# Autodesk Inventor assembly: bike-rack-assembly
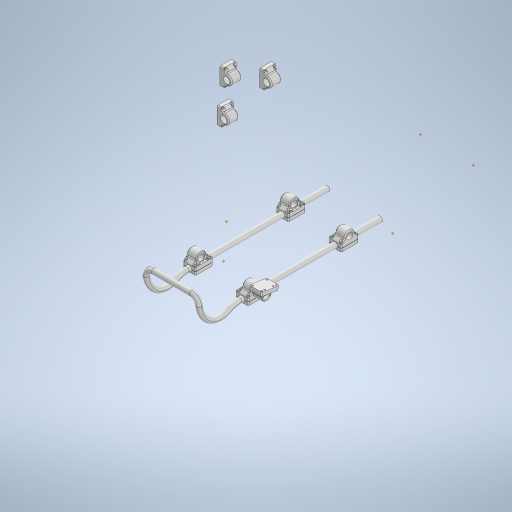
[picture p0: Inventor's stored thumbnail of the model, 512x512]
Saved by Autodesk Inventor 2024.1 (Build 281209000, 209)
## iProperties
Created: 2025-08-15
Part Number: bike-rack-assembly
Document SubType Name: Assembly
Designer: iwheard
Author: iwheard
## Documents named in this file (5)
- C:\Users\iwheard\Documents\0004-CAD\3D-cad-main\bike-rack\bike-rack-assembly.iam
- C:\Users\iwheard\Documents\0004-CAD\3D-cad-main\bike-rack\bike-rack.ipt
- C:\Users\iwheard\Documents\0004-CAD\3D-cad-main\h6-case\rack-mounts.ipt
- C:\Users\iwheard\Documents\0004-CAD\3D-cad-main\h6-case\rack-mounts_MIR.ipt
- C:\Users\iwheard\Documents\0004-CAD\3D-cad-main\h6-case\bucket-mounts.ipt
## Components (9 placed, 4 different names)
1. bike-rack:1 — Flush:1, Mate:1, Flush:2, Tangent:1, Tangent:2
2. rack-mounts:1 — Flush:1, Mate:1, Flush:2, Mate:2, Flush:3, Flush:4, Insert:1, Mate:4
3. rack-mounts:2 — Mate:2, Flush:3, Flush:4
4. rack-mounts_MIR:1 — Flush:5, Flush:6, Mate:3
5. rack-mounts_MIR:2 — Flush:5, Flush:6, Mate:3
6. bucket-mounts:1
7. bucket-mounts:2
8. bucket-mounts:3 — Insert:1, Mate:4
9. bucket-mounts:4
## Relationships (16: Flush 6, Mate 4, Angle 2, Tangent 2, Symmetry 1, Insert 1)
- Flush:1: bike-rack:1 ↔ rack-mounts:1
- Mate:1: bike-rack:1 ↔ rack-mounts:1
- Flush:2 (-240 mm): bike-rack:1 ↔ rack-mounts:1
- Mate:2 (150 mm): rack-mounts:1 ↔ rack-mounts:2
- Flush:3: rack-mounts:1 ↔ rack-mounts:2
- Flush:4: rack-mounts:1 ↔ rack-mounts:2
- Angle:1 (0 deg)
- Tangent:1: bike-rack:1
- Angle:2 (0 deg)
- Tangent:2: bike-rack:1
- Symmetry:1
- Flush:5: rack-mounts_MIR:1 ↔ rack-mounts_MIR:2
- Flush:6: rack-mounts_MIR:1 ↔ rack-mounts_MIR:2
- Mate:3 (150 mm): rack-mounts_MIR:1 ↔ rack-mounts_MIR:2
- Insert:1: rack-mounts:1 ↔ bucket-mounts:3
- Mate:4: rack-mounts:1 ↔ bucket-mounts:3
